# Autodesk Inventor assembly: brazo robot
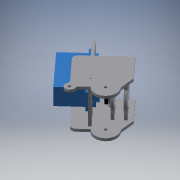
[picture p0: Inventor's stored thumbnail of the model, 180x180]
Saved by Autodesk Inventor 2018 (Build 220112000, 112)
## iProperties
Created: 2020-03-10
Part Number: brazo robot
Material: Genérico
Document SubType Name: Assembly
Designer: sala.ceri
Author: sala.ceri
## Documents named in this file (8)
- C:\Users\david\OneDrive\Documents\robot\ensamble\part7.iam
- C:\Users\david\OneDrive\Documents\robot\piezas\ServoMotor.ipt
- C:\Users\david\OneDrive\Documents\robot\piezas\BaseServo.ipt
- C:\Users\david\OneDrive\Documents\robot\codo2.ipt
- C:\Users\david\OneDrive\Documents\robot\codo.ipt
- C:\Users\david\OneDrive\Documents\robot\cod.ipt
- C:\Users\david\OneDrive\Documents\robot\cod2.ipt
- C:\Users\david\OneDrive\Documents\robot\tapa.ipt
## Components (8 placed, 7 different names)
1. codo:1 — Coincidencia:50, Coincidencia:52, Coincidencia:56, Coincidencia:57
2. codo2:1 — Coincidencia:51, Coincidencia:53, Coincidencia:91
3. cod:1 — Coincidencia:50, Coincidencia:51
4. cod:2 — Coincidencia:52, Coincidencia:53, Coincidencia:91
5. cod2:1 — Coincidencia:56, Coincidencia:57, Coincidencia:58, Coincidencia:60
6. ServoMotor:4 — Coincidencia:58, Coincidencia:60, Coincidencia:61, Coincidencia:62
7. BaseServo:4 — Coincidencia:61, Coincidencia:62, Coincidencia:65, Coincidencia:66, Coincidencia:67
8. tapa:1 — Coincidencia:65, Coincidencia:66, Coincidencia:67
## Relationships (14: Mate 14)
- Coincidencia:50 [Mate]: codo:1 ↔ cod:1
- Coincidencia:51 [Mate]: codo2:1 ↔ cod:1
- Coincidencia:52 [Mate]: codo:1 ↔ cod:2
- Coincidencia:53 [Mate]: codo2:1 ↔ cod:2
- Coincidencia:56 [Mate]: codo:1 ↔ cod2:1
- Coincidencia:57 [Mate]: codo:1 ↔ cod2:1
- Coincidencia:58 [Mate]: cod2:1 ↔ ServoMotor:4
- Coincidencia:60 [Mate]: cod2:1 ↔ ServoMotor:4
- Coincidencia:61 [Mate]: ServoMotor:4 ↔ BaseServo:4
- Coincidencia:62 [Mate]: ServoMotor:4 ↔ BaseServo:4
- Coincidencia:65 [Mate]: BaseServo:4 ↔ tapa:1
- Coincidencia:66 [Mate]: BaseServo:4 ↔ tapa:1
- Coincidencia:67 [Mate]: BaseServo:4 ↔ tapa:1
- Coincidencia:91 [Mate]: codo2:1 ↔ cod:2
